# Autodesk Inventor assembly: Gripper
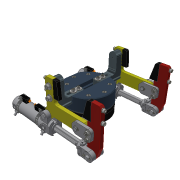
[picture p0: Inventor's stored thumbnail of the model, 180x180]
Saved by Autodesk Inventor 2020.1 (Build 241239000, 239)
## iProperties
Created: 2006-01-31
Part Number: Gripper
Document SubType Name: Assembly
Designer: Kevin
Manufacturer: Standard
Standards Organization: Custom
Weld Material: Default
Author: Kevin
Revision Number: -
## Documents named in this file (12)
- C:\Users\thom_tremblay\Desktop\Inventor ACP Data\Gripper - BOM.iam
- C:\Users\thom_tremblay\Desktop\Inventor ACP Data\Parts\210-100b.ipt
- C:\Users\thom_tremblay\Desktop\Inventor ACP Data\Parts\210-101b.ipt
- C:\Users\thom_tremblay\Desktop\Inventor ACP Data\Content Center\en-US\ISO 4762\M8-65.ipt
- C:\Users\thom_tremblay\Desktop\Inventor ACP Data\Content Center\en-US\ISO 4762\M6-45.ipt
- C:\Users\thom_tremblay\Desktop\Inventor ACP Data\Content Center\en-US\ISO 7089\10.ipt
- C:\Users\thom_tremblay\Desktop\Inventor ACP Data\Assemblies\210-103b.iam
- C:\Users\thom_tremblay\Desktop\Inventor ACP Data\Content Center\en-US\ISO 4762\M8-30.ipt
- C:\Users\thom_tremblay\Desktop\Inventor ACP Data\Assemblies\210-110b.IAM
- C:\Users\thom_tremblay\Desktop\Inventor ACP Data\Parts\210-102 fb.ipt
- C:\Users\thom_tremblay\Desktop\Inventor ACP Data\Assemblies\Actuator.iam
- C:\Users\thom_tremblay\Desktop\Inventor ACP Data\Libraries\Simulation\Gripper_res_{3E676F27-C720-4572-8F7D-DA90B4A1A400}.fres
## Components (32 placed, 10 different names)
1. 210-100b:1 — Mate:1, Insert:1
2. 210-101b:1 — Mate:1, Insert:1, Mate:2, Mate:6, Mate:25, Mate:26, Mate:27, Mate:28, Mate:29, Insert:21, Mate:36, Mate:37, Mate:38, Mate:3
3. 210-102 fb:1 — Mate:2, Mate:3, Insert:36, Angle:3, Mate:42
4. 210-102 fb:2 — Mate:24, Flush:3, Mate:25, Mate:26, Mate:29, Mate:41
5. 210-103b:1 [sub-assembly] — Insert:31, Insert:34, Insert:30, Insert:36
6. 210-103b:2 [sub-assembly] — Mate:24, Flush:3, Insert:26, Insert:35, Insert:27, Insert:37
7. 210-110b:1 [sub-assembly] — Insert:34, Angle:3
8. 210-110b:2 [sub-assembly] — Insert:35, Mate:43
9. Actuator:1 [sub-assembly]
10. Actuator:2 [sub-assembly] — Insert:37, Mate:43
11. ISO 4762 M8 x 45:1 — Mate:6, Insert:22, Mate:42
12. ISO 7089 10 - 140 HV:1 — Insert:22
13. ISO 7089 10 - 140 HV:2 — Insert:23
14. ISO 4762 M8 x 45:2 — Insert:23, Mate:36
15. ISO 7089 10 - 140 HV:3 — Mate:28, Insert:25
16. ISO 4762 M8 x 45:3 — Insert:25, Mate:38
17. ISO 7089 10 - 140 HV:4 — Mate:27, Insert:24
18. ISO 4762 M8 x 45:4 — Mate:37, Insert:24
19. ISO 7089 10 - 140 HV:5 — Insert:33, Insert:30
20. ISO 7089 10 - 140 HV:6 — Insert:31, Insert:32
21. ISO 7089 10 - 140 HV:7 — Insert:26, Insert:28
22. ISO 7089 10 - 140 HV:8 — Insert:29, Insert:27
23. ISO 4762 M8 x 30:1 — Insert:29
24. ISO 4762 M8 x 30:2 — Insert:28, Mate:41
25. ISO 4762 M8 x 30:3 — Insert:32
26. ISO 4762 M8 x 30:4 — Insert:33
27. "ISO 4762 " M8 x 65:1 — Insert:21
28. "ISO 4762 " M8 x 65:2
29. "ISO 4762 " M8 x 65:3
30. "ISO 4762 " M8 x 65:4
31. "ISO 4762 " M8 x 65:5
32. "ISO 4762 " M8 x 65:6
## Component patterns: (8 elements, first: "ISO 4762 " M8 x 65:1)
## Relationships (42: Mate 20, Insert 19, Angle 2, Flush 1)
- Mate:1: 210-100b:1 ↔ 210-101b:1
- Insert:1: 210-100b:1 ↔ 210-101b:1
- Mate:2: 210-101b:1 ↔ 210-102 fb:1
- [Mate]: 210-101b:1 ↔ 210-102 fb:1
- Mate:6: 210-101b:1 ↔ ISO 4762 M8 x 45:1
- [Mate]: 210-102 fb:2 ↔ ISO 7089 10 - 140 HV:1
- [Mate]: 210-101b:1 ↔ ISO 7089 10 - 140 HV:2
- Mate:24: 210-102 fb:2 ↔ 210-103b:2
- Flush:3: 210-102 fb:2 ↔ 210-103b:2
- Mate:25: 210-101b:1 ↔ 210-102 fb:2
- Mate:26: 210-101b:1 ↔ 210-102 fb:2
- Mate:27: 210-101b:1 ↔ ISO 7089 10 - 140 HV:4
- Mate:28: 210-101b:1 ↔ ISO 7089 10 - 140 HV:3
- Mate:29 (30 mm): 210-101b:1 ↔ 210-102 fb:2
- [Insert]: 210-103b:1 ↔ Actuator:1
- Insert:21: 210-101b:1 ↔ "ISO 4762 " M8 x 65:1
- Insert:22: ISO 4762 M8 x 45:1 ↔ ISO 7089 10 - 140 HV:1
- Insert:23: ISO 7089 10 - 140 HV:2 ↔ ISO 4762 M8 x 45:2
- Mate:36: 210-101b:1 ↔ ISO 4762 M8 x 45:2
- Mate:37: 210-101b:1 ↔ ISO 4762 M8 x 45:4
- Insert:24: ISO 7089 10 - 140 HV:4 ↔ ISO 4762 M8 x 45:4
- Insert:25: ISO 7089 10 - 140 HV:3 ↔ ISO 4762 M8 x 45:3
- Mate:38: 210-101b:1 ↔ ISO 4762 M8 x 45:3
- Insert:26: 210-103b:2 ↔ ISO 7089 10 - 140 HV:7
- Insert:28: ISO 7089 10 - 140 HV:7 ↔ ISO 4762 M8 x 30:2
- Insert:29: ISO 7089 10 - 140 HV:8 ↔ ISO 4762 M8 x 30:1
- Insert:31: 210-103b:1 ↔ ISO 7089 10 - 140 HV:6
- Insert:32: ISO 7089 10 - 140 HV:6 ↔ ISO 4762 M8 x 30:3
- Insert:33: ISO 7089 10 - 140 HV:5 ↔ ISO 4762 M8 x 30:4
- Insert:34: 210-103b:1 ↔ 210-110b:1
- Insert:35: 210-103b:2 ↔ 210-110b:2
- [Mate]: 210-110b:1 ↔ Actuator:1
- Insert:27: 210-103b:2 ↔ ISO 7089 10 - 140 HV:8
- Insert:30: 210-103b:1 ↔ ISO 7089 10 - 140 HV:5
- Mate:3: 210-101b:1 ↔ 210-102 fb:1
- Insert:36: 210-102 fb:1 ↔ 210-103b:1
- [Angle] (0 deg): 210-103b:1 ↔ 210-103b:2
- Angle:3 (0 deg): 210-102 fb:1 ↔ 210-110b:1
- Mate:41: 210-102 fb:2 ↔ ISO 4762 M8 x 30:2
- Mate:42: 210-102 fb:1 ↔ ISO 4762 M8 x 45:1
- Insert:37: 210-103b:2 ↔ Actuator:2
- Mate:43: 210-110b:2 ↔ Actuator:2
## Named parameters: sa_0 = -1.46e-11, sa_1 = 14942.9, sa_2 = -1307.34, sa_3 = -1.68e-11, sa_4 = 14942.9, sa_5 = -1307.34, sa_6 = 427.41, sa_7 = -14502, sa_8 = -3809.04, sa_9 = 427.41, sa_10 = -14502, sa_11 = -3809.04, sa_12 = 712.349, sa_13 = -24170, sa_14 = -6348.39, sa_15 = -0, sa_16 = 24904.9, sa_17 = -2178.89
note: some values were not read from the file. Shown as the stored number, unit unknown: "sa_0", "sa_1", "sa_2", "sa_3", "sa_4", "sa_5", "sa_6", "sa_7", "sa_8", "sa_9", "sa_10", "sa_11", "sa_12", "sa_13", "sa_14", "sa_15", "sa_16", "sa_17".
